# Autodesk Inventor assembly: PlanetaryWheel
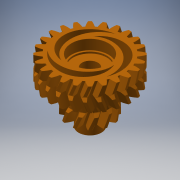
[picture p0: Inventor's stored thumbnail of the model, 180x180]
Saved by Autodesk Inventor 2019.1 (Build 231200000, 200)
## iProperties
Created: 2019-01-01
Part Number: PlanetaryWheel
Material: Generisch
Document SubType Name: Assembly
Designer: JochenAlt
Author: JochenAlt
## Documents named in this file (3)
- D:\Projects\Ondine\CAD\PlanetaryGear2\PlanetaryGearConstruction\PlanetaryWheel.iam
- D:\Projects\Ondine\CAD\PlanetaryGear2\PlanetaryGearConstruction\Stirnzahnrad2-11.ipt
- D:\Projects\Ondine\CAD\PlanetaryGear2\PlanetaryGearConstruction\Stirnzahnrad11.ipt
## Components (2 placed, 1 different names)
1. Stirnzahnrad1:1 — Passend:1, Passend:2
2. Stirnzahnrad1:2 — Passend:1, Passend:2
## Relationships (2: Mate 2)
- Passend:1 [Mate]: Stirnzahnrad1:1 ↔ Stirnzahnrad1:2
- Passend:2 [Mate]: Stirnzahnrad1:1 ↔ Stirnzahnrad1:2
